# Autodesk Inventor assembly: Assembly
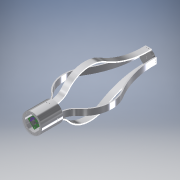
[picture p0: Inventor's stored thumbnail of the model, 180x180]
Saved by Autodesk Inventor 2016 (Build 200138000, 138)
## iProperties
Created: 2016-06-15
Part Number: Assembly
Document SubType Name: Assembly
Designer: Andres
Author: Andres
## Documents named in this file (8)
- Z:\Documents\repositorios\BoreholeCamera\CAD_Probe\Assembly\Assembly.iam
- Z:\Documents\repositorios\BoreholeCamera\CAD_Probe\Enclosure\Parts\Enclosure.ipt
- Z:\Documents\repositorios\BoreholeCamera\CAD_Probe\Camera\Assembly\Assembly.iam
- Z:\Documents\repositorios\BoreholeCamera\CAD_Probe\PCB\STEP\PCB_Probe.iam
- Z:\Documents\repositorios\BoreholeCamera\CAD_Probe\Enclosure\Parts\Cover.ipt
- Z:\Documents\repositorios\BoreholeCamera\CAD_Probe\Shaft Collar\assembly\SSCMN5.iam
- Z:\Documents\repositorios\BoreholeCamera\CAD_Probe\Enclosure\Parts\8inch_Fin.ipt
- Z:\Documents\repositorios\BoreholeCamera\CAD_Probe\Enclosure\Parts\Bottom.ipt
## Components (10 placed, 7 different names)
1. Enclosure:1 — Rigid:1, Rigid:2, Rotational:2, Rotational:3, Rigid:3, Rigid:4, Rigid:5
2. Assembly:1 [sub-assembly] — Rigid:1, Rotational:1
3. PCB_Probe:1 [sub-assembly] — Rotational:1
4. Cover:1 — Rigid:2
5. SSCMN5:1 [sub-assembly] — Rotational:2
6. 8inch_Fin:1 — Rotational:3
7. 8inch_Fin:2 — Rigid:3
8. 8inch_Fin:3 — Rigid:5, Rigid:6
9. 8inch_Fin:4 — Rigid:4
10. Bottom:1 — Rigid:6
## Relationships (9: WeldJoint 6, RevoluteJoint 3)
- Rigid:1 [WeldJoint] (6 mm): Enclosure:1 ↔ Assembly:1
- Rotational:1 [RevoluteJoint] (-20 mm): Assembly:1 ↔ PCB_Probe:1
- Rigid:2 [WeldJoint]: Enclosure:1 ↔ Cover:1
- Rotational:2 [RevoluteJoint]: Enclosure:1 ↔ SSCMN5:1
- Rotational:3 [RevoluteJoint]: Enclosure:1 ↔ 8inch_Fin:1
- Rigid:3 [WeldJoint]: Enclosure:1 ↔ 8inch_Fin:2
- Rigid:4 [WeldJoint]: Enclosure:1 ↔ 8inch_Fin:4
- Rigid:5 [WeldJoint]: Enclosure:1 ↔ 8inch_Fin:3
- Rigid:6 [WeldJoint]: 8inch_Fin:3 ↔ Bottom:1
